# Autodesk Inventor assembly: electronics board frame back
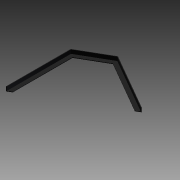
[picture p0: Inventor's stored thumbnail of the model, 180x180]
Saved by Autodesk Inventor 2012 (Build 160160000, 160)
## iProperties
Created: 2011-11-26
Part Number: electronics board frame back
Document SubType Name: Assembly
Designer: Antonella
Author: Antonella
## Documents named in this file (4)
- C:\Users\Antonella\Documents\GCC Robotics 2012 - Mechanical\Robot 2.0\Chassis\electronics board frame back.iam
- C:\Users\Antonella\Documents\GCC Robotics 2012 - Mechanical\Robot 2.0\Chassis\electronics board support side angle.ipt
- C:\Users\Antonella\Documents\GCC Robotics 2012 - Mechanical\Robot 2.0\Chassis\electronics board support side angle_MIR1.ipt
- C:\Users\Antonella\Documents\GCC Robotics 2012 - Mechanical\Robot 2.0\Chassis\electronics board frame back.ipt
## Components (3 placed, 3 different names)
1. electronics board support side angle:1 — Mate:1, Flush:1, Mate:2
2. electronics board support side angle_MIR1:1 — Mate:3, Flush:2, Mate:4
3. electronics board frame back:1 — Mate:1, Flush:1, Mate:2, Mate:3, Flush:2, Mate:4
## Relationships (6: Mate 4, Flush 2)
- Mate:1: electronics board support side angle:1 ↔ electronics board frame back:1
- Flush:1: electronics board support side angle:1 ↔ electronics board frame back:1
- Mate:2: electronics board support side angle:1 ↔ electronics board frame back:1
- Mate:3: electronics board support side angle_MIR1:1 ↔ electronics board frame back:1
- Flush:2: electronics board support side angle_MIR1:1 ↔ electronics board frame back:1
- Mate:4: electronics board support side angle_MIR1:1 ↔ electronics board frame back:1
